# Autodesk Inventor assembly: Complete Roller Pneumatic Cylinder Assembly
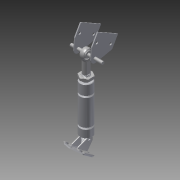
[picture p0: Inventor's stored thumbnail of the model, 180x180]
Saved by Autodesk Inventor 2014 (Build 180170000, 170)
## iProperties
Created: 2014-01-18
Part Number: Complete Roller Pneumatic Cylinder Assembly
Document SubType Name: Assembly
Designer: Michael
Author: Michael
## Documents named in this file (7)
- C:\Users\Michael\Documents\GitHub\2014buildCAD\New Collector\Complete Roller Pneumatic Cylinder Assembly.iam
- C:\Users\Michael\Documents\GitHub\2014buildCAD\New Collector\6498K602 Pneumatic Cylinder Assembly.iam
- C:\Users\Michael\Documents\GitHub\2014buildCAD\New Collector\Axle 0.190 in 3 in length.ipt
- C:\Users\Michael\Documents\GitHub\2014buildCAD\New Collector\Bracket.ipt
- C:\Users\Michael\Documents\GitHub\2014buildCAD\New Collector\Rod End (McMaster Part #6498K592).ipt
- C:\Users\Michael\Documents\GitHub\2014buildCAD\New Collector\Roller Pneumatic Back Connector (Custom).ipt
- C:\Users\Michael\Documents\GitHub\2014buildCAD\New Collector\Foot Bracket Mount (McMaster Part #6498K710).ipt
## Components (7 placed, 6 different names)
1. 6498K602 Pneumatic Cylinder Assembly:1 [sub-assembly] — Mate:1, Mate:3, Mate:4, Mate:14
2. Axle 0.190 in 3 in length:1 — Mate:5, Mate:15, Mate:16, Flush:1
3. Rod End (McMaster Part #6498K592):1 — Mate:1, Mate:5, Mate:14, Mate:19
4. Roller Pneumatic Back Connector (Custom):1 — Mate:11, Mate:12, Mate:13
5. Foot Bracket Mount (McMaster Part #6498K710):1 — Mate:3, Mate:4, Mate:11, Mate:12, Mate:13
6. Bracket:2 — Mate:15, Mate:17, Mate:18
7. Bracket:3 — Mate:16, Mate:17, Mate:18, Mate:19, Flush:1
## Relationships (14: Mate 13, Flush 1)
- Mate:1: 6498K602 Pneumatic Cylinder Assembly:1 ↔ Rod End (McMaster Part #6498K592):1
- Mate:3: 6498K602 Pneumatic Cylinder Assembly:1 ↔ Foot Bracket Mount (McMaster Part #6498K710):1
- Mate:4: 6498K602 Pneumatic Cylinder Assembly:1 ↔ Foot Bracket Mount (McMaster Part #6498K710):1
- Mate:5: Axle 0.190 in 3 in length:1 ↔ Rod End (McMaster Part #6498K592):1
- Mate:11: Roller Pneumatic Back Connector (Custom):1 ↔ Foot Bracket Mount (McMaster Part #6498K710):1
- Mate:12: Roller Pneumatic Back Connector (Custom):1 ↔ Foot Bracket Mount (McMaster Part #6498K710):1
- Mate:13: Roller Pneumatic Back Connector (Custom):1 ↔ Foot Bracket Mount (McMaster Part #6498K710):1
- Mate:14: 6498K602 Pneumatic Cylinder Assembly:1 ↔ Rod End (McMaster Part #6498K592):1
- Mate:15: Axle 0.190 in 3 in length:1 ↔ Bracket:2
- Mate:16: Axle 0.190 in 3 in length:1 ↔ Bracket:3
- Mate:17 (25.4 mm): Bracket:2 ↔ Bracket:3
- Mate:18: Bracket:2 ↔ Bracket:3
- Mate:19 (8.7376 mm): Rod End (McMaster Part #6498K592):1 ↔ Bracket:3
- Flush:1 (-9.525 mm): Axle 0.190 in 3 in length:1 ↔ Bracket:3
